# Autodesk Inventor assembly: EnsambleCajaVariadores
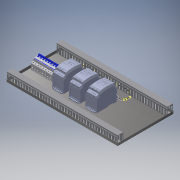
[picture p0: Inventor's stored thumbnail of the model, 180x180]
Saved by Autodesk Inventor 2017 (Build 210142000, 142)
## iProperties
Created: 2021-02-22
Part Number: EnsambleCajaVariadores
Document SubType Name: Assembly
Designer: USUARIO
Author: USUARIO
## Documents named in this file (7)
- D:\Laboratorio\Modulo Flujo Laminar\2021\JPCFLVMOD-2PM TOUCH Abaco OP202130 #0045884XX\Modelo\EnsambleCajaVariadores.iam
- D:\Laboratorio\Modulo Flujo Laminar\2021\JPCFLVMOD-2PM TOUCH Abaco OP202130 #0045884XX\Modelo\BANDEJA VARIADORES CPM-200-2021.ipt
- D:\Laboratorio\Modulo Flujo Laminar\2021\JPCFLVMOD-2PM TOUCH Abaco OP202130 #0045884XX\Modelo\E3 S1 Plastic Set1.ipt
- C:\Users\USUARIO\Documents\Inventor\Canaleta 40x60 800mm.iam
- D:\Laboratorio\Modulo Flujo Laminar\2021\JPCFLVMOD-2PM TOUCH Abaco OP202130 #0045884XX\Modelo\Riel120mm.ipt
- D:\Laboratorio\Modulo Flujo Laminar\2021\JPCFLVMOD-2PM TOUCH Abaco OP202130 #0045884XX\Modelo\EnsambleCajaVariadores\AIP\Cable and Harness\EnsambleCajaVariadores.Harness1.iam
- C:\Modelos 3D y DXF\B1A-NOARK.stp\disjuntor weg - mdw c10.ipt
## Components (11 placed, 6 different names)
1. BANDEJA VARIADORES CPM-200-2021:1 — Mate:2, Mate:3, Mate:4, Mate:5, Mate:6, Mate:7, Mate:10, Mate:11, Insert:1, Insert:2, Insert:3
2. E3 S1 Plastic Set1:1 — Insert:2
3. Canaleta 40x60 800mm:1 [sub-assembly] — Mate:3, Mate:4, Mate:6, Mate:12
4. Canaleta 40x60 800mm:2 [sub-assembly] — Mate:2, Mate:5, Mate:7
5. E3 S1 Plastic Set1:2 — Insert:1
6. E3 S1 Plastic Set1:3 — Insert:3
7. Riel120mm:1 — Mate:10, Mate:11, Mate:12, Mate:13, Mate:14, Mate:15, Mate:16, Mate:17, Mate:18
8. Harness1 [sub-assembly]
9. disjuntor weg - mdw c10:1 — Mate:13, Mate:14
10. disjuntor weg - mdw c10:2 — Mate:16, Mate:18
11. disjuntor weg - mdw c10:3 — Mate:15, Mate:17
## Relationships (18: Mate 15, Insert 3)
- Mate:2: BANDEJA VARIADORES CPM-200-2021:1 ↔ Canaleta 40x60 800mm:2
- Mate:3: BANDEJA VARIADORES CPM-200-2021:1 ↔ Canaleta 40x60 800mm:1
- Mate:4 (0.5 mm): BANDEJA VARIADORES CPM-200-2021:1 ↔ Canaleta 40x60 800mm:1
- Mate:5 (0.5 mm): BANDEJA VARIADORES CPM-200-2021:1 ↔ Canaleta 40x60 800mm:2
- Mate:6 (1 mm): BANDEJA VARIADORES CPM-200-2021:1 ↔ Canaleta 40x60 800mm:1
- Mate:7 (1 mm): BANDEJA VARIADORES CPM-200-2021:1 ↔ Canaleta 40x60 800mm:2
- Mate:10: BANDEJA VARIADORES CPM-200-2021:1 ↔ Riel120mm:1
- Mate:11 (5 mm): BANDEJA VARIADORES CPM-200-2021:1 ↔ Riel120mm:1
- Mate:12 (159 mm): Canaleta 40x60 800mm:1 ↔ Riel120mm:1
- Insert:1: BANDEJA VARIADORES CPM-200-2021:1 ↔ E3 S1 Plastic Set1:2
- Insert:2: BANDEJA VARIADORES CPM-200-2021:1 ↔ E3 S1 Plastic Set1:1
- Insert:3: BANDEJA VARIADORES CPM-200-2021:1 ↔ E3 S1 Plastic Set1:3
- Mate:13: Riel120mm:1 ↔ disjuntor weg - mdw c10:1
- Mate:14: Riel120mm:1 ↔ disjuntor weg - mdw c10:1
- Mate:15: Riel120mm:1 ↔ disjuntor weg - mdw c10:3
- Mate:16: Riel120mm:1 ↔ disjuntor weg - mdw c10:2
- Mate:17: Riel120mm:1 ↔ disjuntor weg - mdw c10:3
- Mate:18: Riel120mm:1 ↔ disjuntor weg - mdw c10:2
